# Autodesk Inventor assembly: Ensamblaje carcasa superior
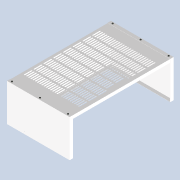
[picture p0: Inventor's stored thumbnail of the model, 180x180]
Saved by Autodesk Inventor 2021 (Build 250183000, 183)
## iProperties
Created: 2021-04-15
Part Number: Ensamblaje carcasa superior
Document SubType Name: Assembly
Designer: Admin
Mass: 3693.67 g
Surface Area: 11669.8 cm^2
Volume: 469.216 cm^3
Density: 7.872 g/cm^3
Author: Admin
## Documents named in this file (7)
- E:\Documentos\Documentos\Michael_Rodriguez\Universidad_Nacional\Doceaba matricula\PAI\Proyecto PAI\Proyecto_PAI_2021\01 CAD\Ensamblaje carcasa superior.iam
- E:\Documentos\Documentos\Michael_Rodriguez\Universidad_Nacional\Doceaba matricula\PAI\Proyecto PAI\Proyecto_PAI_2021\01 CAD\Tapa_superior_superior.ipt
- E:\Documentos\Documentos\Michael_Rodriguez\Universidad_Nacional\Doceaba matricula\PAI\Proyecto PAI\Proyecto_PAI_2021\01 CAD\Tapa_superior_izquierda.ipt
- E:\Documentos\Documentos\Michael_Rodriguez\Universidad_Nacional\Doceaba matricula\PAI\Proyecto PAI\Proyecto_PAI_2021\01 CAD\Tapa_superior_derecha.ipt
- E:\Documentos\Documentos\Michael_Rodriguez\Universidad_Nacional\Doceaba matricula\PAI\Proyecto PAI\Proyecto_PAI_2021\01 CAD\ISO 7380-1 - M5 x 8.ipt
- E:\Documentos\Documentos\Michael_Rodriguez\Universidad_Nacional\Doceaba matricula\PAI\Proyecto PAI\Proyecto_PAI_2021\01 CAD\BS 4320 - M5 (Forma A).ipt
- E:\Documentos\Documentos\Michael_Rodriguez\Universidad_Nacional\Doceaba matricula\PAI\Proyecto PAI\Proyecto_PAI_2021\01 CAD\BS 4183 - M5(1).ipt
## Components (33 placed, 6 different names)
1. Tapa_superior_superior:1 — Coincidencia:1, Coincidencia:2, Coincidencia:3, Coincidencia:4, Coincidencia:5, Coincidencia:6, De rotación:23, De rotación:24, De rotación:25, De rotación:26, De rotación:27, De rotación:28, De rotación:29, De rotación:30, De rotación:31, De rotación:32
2. Tapa_superior_izquierda:1 — Coincidencia:1, Coincidencia:2, Coincidencia:3, De rotación:5, De rotación:6, De rotación:7, De rotación:10, De rotación:11
3. Tapa_superior_derecha:1 — Coincidencia:4, Coincidencia:5, Coincidencia:6, De rotación:1, De rotación:3, De rotación:4, De rotación:8, De rotación:9
4. ISO 7380-1 M5 x 8:1 — De rotación:2
5. ISO 7380-1 M5 x 8:3 — De rotación:15
6. ISO 7380-1 M5 x 8:4 — De rotación:12
7. ISO 7380-1 M5 x 8:5 — De rotación:13
8. ISO 7380-1 M5 x 8:6 — De rotación:14
9. ISO 7380-1 M5 x 8:7 — De rotación:18
10. ISO 7380-1 M5 x 8:8 — De rotación:19
11. ISO 7380-1 M5 x 8:9 — De rotación:16
12. ISO 7380-1 M5 x 8:10 — De rotación:17
13. BS 4320 Forma AB M5 (Forma A):1 — De rotación:3, De rotación:15
14. BS 4320 Forma AB M5 (Forma A):2 — De rotación:1, De rotación:2
15. BS 4320 Forma AB M5 (Forma A):3 — De rotación:4, De rotación:20
16. BS 4320 Forma AB M5 (Forma A):4 — De rotación:5, De rotación:12
17. BS 4320 Forma AB M5 (Forma A):5 — De rotación:7, De rotación:14
18. BS 4320 Forma AB M5 (Forma A):6 — De rotación:6, De rotación:13
19. BS 4320 Forma AB M5 (Forma A):7 — De rotación:8, De rotación:18
20. BS 4320 Forma AB M5 (Forma A):8 — De rotación:9, De rotación:19
21. BS 4320 Forma AB M5 (Forma A):9 — De rotación:10, De rotación:16
22. BS 4320 Forma AB M5 (Forma A):10 — De rotación:11, De rotación:17
23. ISO 7380-1 M5 x 8:11 — De rotación:20
24. BS 4183 - Métrico M5:1 — De rotación:23
25. BS 4183 - Métrico M5:2 — De rotación:25
26. BS 4183 - Métrico M5:3 — De rotación:24
27. BS 4183 - Métrico M5:4 — De rotación:26
28. BS 4183 - Métrico M5:5 — De rotación:27
29. BS 4183 - Métrico M5:6 — De rotación:28
30. BS 4183 - Métrico M5:7 — De rotación:29
31. BS 4183 - Métrico M5:8 — De rotación:30
32. BS 4183 - Métrico M5:9 — De rotación:31
33. BS 4183 - Métrico M5:10 — De rotación:32
## Relationships (36: RevoluteJoint 30, Mate 6)
- Coincidencia:1 [Mate]: Tapa_superior_superior:1 ↔ Tapa_superior_izquierda:1
- Coincidencia:2 [Mate]: Tapa_superior_superior:1 ↔ Tapa_superior_izquierda:1
- Coincidencia:3 [Mate]: Tapa_superior_superior:1 ↔ Tapa_superior_izquierda:1
- Coincidencia:4 [Mate]: Tapa_superior_superior:1 ↔ Tapa_superior_derecha:1
- Coincidencia:5 [Mate]: Tapa_superior_superior:1 ↔ Tapa_superior_derecha:1
- Coincidencia:6 [Mate]: Tapa_superior_superior:1 ↔ Tapa_superior_derecha:1
- De rotación:1 [RevoluteJoint]: Tapa_superior_derecha:1 ↔ BS 4320 Forma AB M5 (Forma A):2
- De rotación:2 [RevoluteJoint]: ISO 7380-1 M5 x 8:1 ↔ BS 4320 Forma AB M5 (Forma A):2
- De rotación:3 [RevoluteJoint]: Tapa_superior_derecha:1 ↔ BS 4320 Forma AB M5 (Forma A):1
- De rotación:4 [RevoluteJoint]: Tapa_superior_derecha:1 ↔ BS 4320 Forma AB M5 (Forma A):3
- De rotación:5 [RevoluteJoint]: Tapa_superior_izquierda:1 ↔ BS 4320 Forma AB M5 (Forma A):4
- De rotación:6 [RevoluteJoint]: Tapa_superior_izquierda:1 ↔ BS 4320 Forma AB M5 (Forma A):6
- De rotación:7 [RevoluteJoint]: Tapa_superior_izquierda:1 ↔ BS 4320 Forma AB M5 (Forma A):5
- De rotación:8 [RevoluteJoint]: Tapa_superior_derecha:1 ↔ BS 4320 Forma AB M5 (Forma A):7
- De rotación:9 [RevoluteJoint]: Tapa_superior_derecha:1 ↔ BS 4320 Forma AB M5 (Forma A):8
- De rotación:10 [RevoluteJoint]: Tapa_superior_izquierda:1 ↔ BS 4320 Forma AB M5 (Forma A):9
- De rotación:11 [RevoluteJoint]: Tapa_superior_izquierda:1 ↔ BS 4320 Forma AB M5 (Forma A):10
- De rotación:12 [RevoluteJoint]: ISO 7380-1 M5 x 8:4 ↔ BS 4320 Forma AB M5 (Forma A):4
- De rotación:13 [RevoluteJoint]: ISO 7380-1 M5 x 8:5 ↔ BS 4320 Forma AB M5 (Forma A):6
- De rotación:14 [RevoluteJoint]: ISO 7380-1 M5 x 8:6 ↔ BS 4320 Forma AB M5 (Forma A):5
- De rotación:15 [RevoluteJoint]: ISO 7380-1 M5 x 8:3 ↔ BS 4320 Forma AB M5 (Forma A):1
- De rotación:16 [RevoluteJoint]: ISO 7380-1 M5 x 8:9 ↔ BS 4320 Forma AB M5 (Forma A):9
- De rotación:17 [RevoluteJoint]: ISO 7380-1 M5 x 8:10 ↔ BS 4320 Forma AB M5 (Forma A):10
- De rotación:18 [RevoluteJoint]: ISO 7380-1 M5 x 8:7 ↔ BS 4320 Forma AB M5 (Forma A):7
- De rotación:19 [RevoluteJoint]: ISO 7380-1 M5 x 8:8 ↔ BS 4320 Forma AB M5 (Forma A):8
- De rotación:20 [RevoluteJoint]: BS 4320 Forma AB M5 (Forma A):3 ↔ ISO 7380-1 M5 x 8:11
- De rotación:23 [RevoluteJoint]: Tapa_superior_superior:1 ↔ BS 4183 - Métrico M5:1
- De rotación:24 [RevoluteJoint]: Tapa_superior_superior:1 ↔ BS 4183 - Métrico M5:3
- De rotación:25 [RevoluteJoint]: Tapa_superior_superior:1 ↔ BS 4183 - Métrico M5:2
- De rotación:26 [RevoluteJoint]: Tapa_superior_superior:1 ↔ BS 4183 - Métrico M5:4
- De rotación:27 [RevoluteJoint]: Tapa_superior_superior:1 ↔ BS 4183 - Métrico M5:5
- De rotación:28 [RevoluteJoint]: Tapa_superior_superior:1 ↔ BS 4183 - Métrico M5:6
- De rotación:29 [RevoluteJoint]: Tapa_superior_superior:1 ↔ BS 4183 - Métrico M5:7
- De rotación:30 [RevoluteJoint]: Tapa_superior_superior:1 ↔ BS 4183 - Métrico M5:8
- De rotación:31 [RevoluteJoint]: Tapa_superior_superior:1 ↔ BS 4183 - Métrico M5:9
- De rotación:32 [RevoluteJoint]: Tapa_superior_superior:1 ↔ BS 4183 - Métrico M5:10
